# Autodesk Inventor assembly: cam_holder
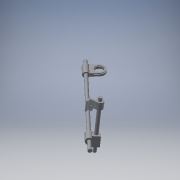
[picture p0: Inventor's stored thumbnail of the model, 180x180]
Saved by Autodesk Inventor 2019 (Build 230136000, 136)
## iProperties
Created: 2024-08-06
Part Number: cam_holder
Material: Generisch
Document SubType Name: Assembly
Designer: nic
Author: nic
## Documents named in this file (7)
- C:\Users\Nicolas Frick\Sync\OneDrive\wtm\nicol_rh8d\atxmega_qenc\inventor\cam_holder.iam
- C:\Users\Nicolas Frick\Sync\OneDrive\wtm\nicol_rh8d\atxmega_qenc\inventor\cam_holder_wrist_part.ipt
- C:\Users\Nicolas Frick\Sync\OneDrive\wtm\nicol_rh8d\atxmega_qenc\inventor\pipe_700.ipt
- C:\Users\Nicolas Frick\Sync\OneDrive\wtm\nicol_rh8d\atxmega_qenc\inventor\pipe_300.ipt
- C:\Users\Nicolas Frick\Sync\OneDrive\wtm\nicol_rh8d\atxmega_qenc\inventor\cam_holder_angle_part.ipt
- C:\Users\Nicolas Frick\Sync\OneDrive\wtm\nicol_rh8d\atxmega_qenc\inventor\cam_holder_end_part.ipt
- C:\Users\Nicolas Frick\Sync\OneDrive\wtm\nicol_rh8d\atxmega_qenc\inventor\cam_holder_hog_part.ipt
## Components (6 placed, 6 different names)
1. cam_holder_wrist_part:1 — Passend:1, Passend:2, Passend:3
2. pipe_700:1 — Passend:3, Passend:4
3. pipe_300:1 — Passend:5, Passend:6
4. cam_holder_angle_part:1 — Passend:4, Passend:5
5. cam_holder_end_part:1 — Passend:6, Passend:7, Passend:8
6. cam_holder_hog_part:1 — Passend:7, Passend:8
## Relationships (8: Mate 8)
- Passend:1 [Mate]: cam_holder_wrist_part:1
- Passend:2 [Mate]: cam_holder_wrist_part:1
- Passend:3 [Mate]: cam_holder_wrist_part:1 ↔ pipe_700:1
- Passend:4 [Mate]: pipe_700:1 ↔ cam_holder_angle_part:1
- Passend:5 [Mate]: pipe_300:1 ↔ cam_holder_angle_part:1
- Passend:6 [Mate]: pipe_300:1 ↔ cam_holder_end_part:1
- Passend:7 [Mate]: cam_holder_end_part:1 ↔ cam_holder_hog_part:1
- Passend:8 [Mate]: cam_holder_end_part:1 ↔ cam_holder_hog_part:1
